# Autodesk Inventor assembly: WheelAssembly
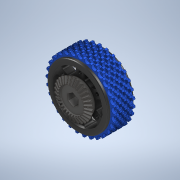
[picture p0: Inventor's stored thumbnail of the model, 180x180]
Saved by Autodesk Inventor 2020 (Build 240168000, 168)
## iProperties
Created: 2019-07-10
Part Number: WheelAssembly
Document SubType Name: Assembly
Designer: Connor
Author: Connor
## Documents named in this file (5)
- C:\Users\Connor\Documents\GrabCAD\2019 Robot\Swerve\TorqyoDriftV2\3inVariant\WheelAssembly.iam
- C:\Users\Connor\Documents\GrabCAD\2019 Robot\Swerve\TorqyoDriftV2\3inVariant\3inWheelHalf.ipt
- C:\Users\Connor\Documents\GrabCAD\2019 Robot\Swerve\TorqyoDriftV2\3inVariant\HubPlate.ipt
- C:\Users\Connor\Documents\GrabCAD\2019 Robot\Swerve\TorqyoDriftV2\3inVariant\3inBlueTread.ipt
- C:\Users\Connor\Documents\GrabCAD\2019 Robot\Swerve\TorqyoDriftV2\Bevel30t.ipt
## Components (6 placed, 4 different names)
1. 3inWheelHalf:1 — Insert:1, Mate:1, Insert:3, Mate:3
2. HubPlate:1 — Insert:1, Mate:1, Insert:2, Mate:2
3. 3inWheelHalf:2 — Insert:2, Mate:2, Mate:4
4. 3inBlueTread:1 — Insert:3
5. Bevel30t:1 — Mate:3, Mate:5
6. Bevel30t:2 — Mate:4, Mate:5
## Relationships (8: Mate 5, Insert 3)
- Insert:1: 3inWheelHalf:1 ↔ HubPlate:1
- Mate:1: 3inWheelHalf:1 ↔ HubPlate:1
- Insert:2: HubPlate:1 ↔ 3inWheelHalf:2
- Mate:2: HubPlate:1 ↔ 3inWheelHalf:2
- Insert:3: 3inWheelHalf:1 ↔ 3inBlueTread:1
- Mate:3: 3inWheelHalf:1 ↔ Bevel30t:1
- Mate:4: 3inWheelHalf:2 ↔ Bevel30t:2
- Mate:5 (10.9474 mm): Bevel30t:1 ↔ Bevel30t:2
